# Autodesk Inventor assembly: S8x4
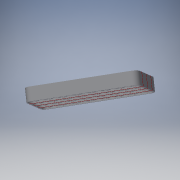
[picture p0: Inventor's stored thumbnail of the model, 180x180]
Saved by Autodesk Inventor 2019 (Build 230136000, 136)
## iProperties
Created: 2019-01-31
Part Number: S8x4
Document SubType Name: Assembly
Designer: Varga Daniel
Author: Varga Daniel
## Documents named in this file (7)
- C:\!_Dani\!_cloud\OneDrive\!_munka\Revolution\RevvyDemoKit\Structural parts\Straight Beams\S3+x4.iam
- C:\!_Dani\!_cloud\OneDrive\!_munka\Revolution\RevvyDemoKit\Structural parts\Straight Beams\straight_beam_side_part.ipt
- C:\!_Dani\!_cloud\OneDrive\!_munka\Revolution\RevvyDemoKit\Structural parts\Straight Beams\straight_beam_inner_part.ipt
- C:\!_Dani\!_cloud\OneDrive\!_munka\Revolution\RevvyDemoKit\Structural parts\Straight Beams\straight_beam_corner_part.ipt
- C:\!_Dani\!_cloud\OneDrive\!_munka\Revolution\RevvyDemoKit\Structural parts\Straight Beams\straight_beam_top_bot_part.ipt
- S4x4.iam
- S8x4.iam
## Components (32 placed, 4 different names)
1. straight_beam_corner_part:1 — Flush:1, Flush:2, Mate:1, Flush:3, Flush:4, Mate:2, Flush:5, Flush:6, Flush:11, Flush:12, Mate:5, Mate:8
2. straight_beam_corner_part:2 — Mate:1, Flush:3, Flush:4
3. straight_beam_corner_part:3 — Flush:11, Flush:12, Mate:5, Flush:13, Flush:14, Mate:6, Flush:15, Flush:16, Mate:7
4. straight_beam_corner_part:4 — Flush:13, Flush:14, Mate:6
5. straight_beam_top_bot_part:1 — Flush:1, Flush:2, Mate:2
6. straight_beam_top_bot_part:2
7. straight_beam_top_bot_part:3 — Flush:15, Flush:16, Mate:7
8. straight_beam_top_bot_part:4
9. straight_beam_side_part:2 — Flush:7, Flush:8, Mate:3
10. straight_beam_side_part:1 — Flush:5, Flush:6, Flush:7, Flush:8, Mate:3, Flush:9, Flush:10, Mate:4, Mate:8
11. straight_beam_side_part:3
12. straight_beam_side_part:4
13. straight_beam_side_part:5
14. straight_beam_side_part:6
15. straight_beam_side_part:7
16. straight_beam_side_part:8
17. straight_beam_side_part:9
18. straight_beam_side_part:10
19. straight_beam_side_part:11
20. straight_beam_side_part:12
21. straight_beam_inner_part:1 — Flush:9, Flush:10, Mate:4
22. straight_beam_inner_part:2
23. straight_beam_inner_part:3
24. straight_beam_inner_part:4
25. straight_beam_inner_part:5
26. straight_beam_inner_part:6
27. straight_beam_inner_part:7
28. straight_beam_inner_part:8
29. straight_beam_inner_part:9
30. straight_beam_inner_part:10
31. straight_beam_inner_part:11
32. straight_beam_inner_part:12
## Component patterns: (2 elements, first: straight_beam_top_bot_part:1), (2 elements, first: straight_beam_top_bot_part:3), (6 elements, first: straight_beam_side_part:2 + straight_beam_side_part:1), (2 elements, first: straight_beam_inner_part:1), Component Pattern 6:2 (2 elements), Component Pattern 6:3 (2 elements), Component Pattern 6:4 (2 elements), Component Pattern 6:5 (2 elements), Component Pattern 6:6 (2 elements)
## Relationships (24: Flush 16, Mate 8)
- Flush:1: straight_beam_corner_part:1 ↔ straight_beam_top_bot_part:1
- Flush:2: straight_beam_corner_part:1 ↔ straight_beam_top_bot_part:1
- Mate:1 (20 mm): straight_beam_corner_part:1 ↔ straight_beam_corner_part:2
- Flush:3: straight_beam_corner_part:1 ↔ straight_beam_corner_part:2
- Flush:4: straight_beam_corner_part:1 ↔ straight_beam_corner_part:2
- Mate:2: straight_beam_corner_part:1 ↔ straight_beam_top_bot_part:1
- Flush:5: straight_beam_corner_part:1 ↔ straight_beam_side_part:1
- Flush:6: straight_beam_corner_part:1 ↔ straight_beam_side_part:1
- Flush:7: straight_beam_side_part:2 ↔ straight_beam_side_part:1
- Flush:8: straight_beam_side_part:2 ↔ straight_beam_side_part:1
- Mate:3 (20 mm): straight_beam_side_part:2 ↔ straight_beam_side_part:1
- Flush:9: straight_beam_side_part:1 ↔ straight_beam_inner_part:1
- Flush:10: straight_beam_side_part:1 ↔ straight_beam_inner_part:1
- Mate:4: straight_beam_side_part:1 ↔ straight_beam_inner_part:1
- Flush:11: straight_beam_corner_part:1 ↔ straight_beam_corner_part:3
- Flush:12: straight_beam_corner_part:1 ↔ straight_beam_corner_part:3
- Mate:5 (60 mm): straight_beam_corner_part:1 ↔ straight_beam_corner_part:3
- Flush:13: straight_beam_corner_part:3 ↔ straight_beam_corner_part:4
- Flush:14: straight_beam_corner_part:3 ↔ straight_beam_corner_part:4
- Mate:6 (20 mm): straight_beam_corner_part:3 ↔ straight_beam_corner_part:4
- Flush:15: straight_beam_corner_part:3 ↔ straight_beam_top_bot_part:3
- Flush:16: straight_beam_corner_part:3 ↔ straight_beam_top_bot_part:3
- Mate:7: straight_beam_corner_part:3 ↔ straight_beam_top_bot_part:3
- Mate:8: straight_beam_corner_part:1 ↔ straight_beam_side_part:1
